# Autodesk Inventor assembly: Rotor
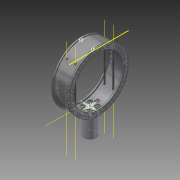
[picture p0: Inventor's stored thumbnail of the model, 180x180]
Saved by Autodesk Inventor 2013 (Build 170138000, 138)
## iProperties
Created: 2012-12-21
Part Number: Rotor
Document SubType Name: Assembly
Designer: Lukas
Author: Lukas
## Documents named in this file (5)
- C:\Users\Lukas\Documents\12 Klasse\Seminarkurs\Rotor\Rotor.iam
- C:\Users\Lukas\Documents\12 Klasse\Seminarkurs\Rotor\Rotorkopf.ipt
- C:\Users\Lukas\Documents\12 Klasse\Seminarkurs\Rotor\Gewindestange3.ipt
- C:\Users\Lukas\Documents\12 Klasse\Seminarkurs\Rotor\Achse.ipt
- C:\Users\Lukas\Documents\12 Klasse\Seminarkurs\Rotor\Rotor\Konstruktions-Assistent\Schraubenverbindung7.iam
## Components (7 placed, 4 different names)
1. Rotorkopf:1 — Passend:7, Passend:8, Passend:9, Passend:10, Fluchtend:1, Fluchtend:2, Fluchtend:3, Fluchtend:4, Passend:11, Passend:12, Passend:13, Passend:14, Passend:15
2. Gewindestange3:1 — Passend:7, Fluchtend:2
3. Gewindestange3:2 — Passend:8, Fluchtend:1
4. Gewindestange3:3 — Passend:9, Fluchtend:3
5. Gewindestange3:4 — Passend:10, Fluchtend:4
6. Achse:1 — Passend:11, Passend:12, Passend:13
7. Schraubenverbindung:1 [sub-assembly] — Passend:14, Passend:15
## Relationships (13: Mate 9, Flush 4)
- Passend:7 [Mate]: Rotorkopf:1 ↔ Gewindestange3:1
- Passend:8 [Mate]: Rotorkopf:1 ↔ Gewindestange3:2
- Passend:9 [Mate]: Rotorkopf:1 ↔ Gewindestange3:3
- Passend:10 [Mate]: Rotorkopf:1 ↔ Gewindestange3:4
- Fluchtend:1 [Flush] (30 mm): Rotorkopf:1 ↔ Gewindestange3:2
- Fluchtend:2 [Flush] (30 mm): Rotorkopf:1 ↔ Gewindestange3:1
- Fluchtend:3 [Flush] (30 mm): Rotorkopf:1 ↔ Gewindestange3:3
- Fluchtend:4 [Flush] (30 mm): Rotorkopf:1 ↔ Gewindestange3:4
- Passend:11 [Mate]: Rotorkopf:1 ↔ Achse:1
- Passend:12 [Mate]: Rotorkopf:1 ↔ Achse:1
- Passend:13 [Mate]: Rotorkopf:1 ↔ Achse:1
- Passend:14 [Mate]: Rotorkopf:1 ↔ Schraubenverbindung:1
- Passend:15 [Mate]: Rotorkopf:1 ↔ Schraubenverbindung:1
